# Autodesk Inventor assembly: Chassisv1
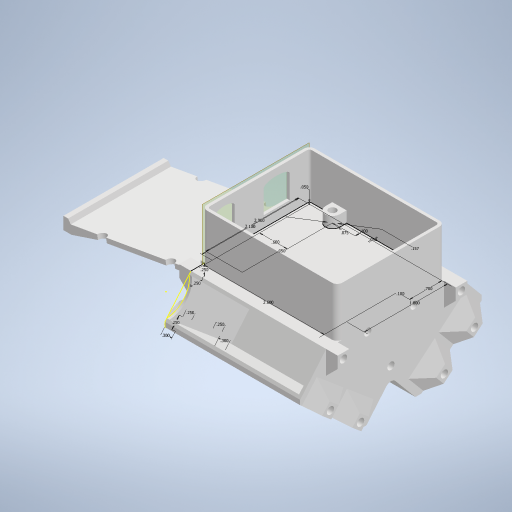
[picture p0: Inventor's stored thumbnail of the model, 512x512]
Saved by Autodesk Inventor 2023 (Build 270158030, 158C)
## iProperties
Created: 2024-03-25
Part Number: Chassisv1
Document SubType Name: Assembly
Designer: lvrectanus0
Author: lvrectanus0
## Documents named in this file (4)
- C:\Users\lvrectanus0\Documents\Github\SPARKLabs-ArduinoProjects\project\CAD\Autodesk\Chassisv1.iam
- C:\Users\lvrectanus0\Documents\Github\SPARKLabs-ArduinoProjects\project\CAD\Autodesk\ArduinoHolder-v2.ipt
- C:\Users\lvrectanus0\Documents\Github\SPARKLabs-ArduinoProjects\project\CAD\Autodesk\BatterMountv1.ipt
- C:\Users\lvrectanus0\Documents\Github\SPARKLabs-ArduinoProjects\project\CAD\Autodesk\BreadboardHolderv1.ipt
## Components (3 placed, 3 different names)
1. ArduinoHolder-v2:1 — Flush:1, Flush:2
2. BatterMountv1:1 — Flush:1, Flush:2, Flush:3
3. BreadboardHolderv1:1 — Flush:3
## Relationships (3: Flush 3)
- Flush:1: ArduinoHolder-v2:1 ↔ BatterMountv1:1
- Flush:2: ArduinoHolder-v2:1 ↔ BatterMountv1:1
- Flush:3: BatterMountv1:1 ↔ BreadboardHolderv1:1
